# Autodesk Inventor assembly: Inner_Components
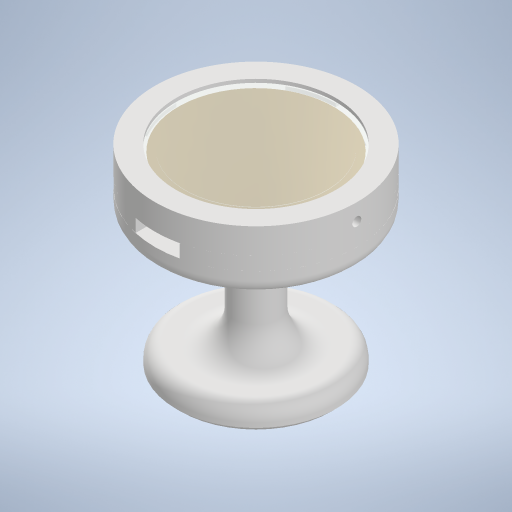
[picture p0: Inventor's stored thumbnail of the model, 512x512]
Saved by Autodesk Inventor 2023 (Build 270158000, 158)
## iProperties
Created: 2023-02-27
Part Number: Inner_Components
Document SubType Name: Assembly
Designer: maste
Author: maste
## Documents named in this file (6)
- C:\Users\maste\Documents\GitHub\Remote-Stethoscope\3D_models\ThonkLabs 1ne\Inner_Components.iam
- C:\Users\maste\Documents\GitHub\Remote-Stethoscope\3D_models\ThonkLabs 1ne\PiezoMount.ipt
- C:\Users\maste\Documents\GitHub\Remote-Stethoscope\3D_models\ThonkLabs 1ne\Piezo.ipt
- C:\Users\maste\Documents\GitHub\Remote-Stethoscope\3D_models\ThonkLabs 1ne\Diaphragm.ipt
- C:\Users\maste\Documents\GitHub\Remote-Stethoscope\3D_models\ThonkLabs 1ne\Diaphragm_lock.ipt
- C:\Users\maste\Documents\GitHub\Remote-Stethoscope\3D_models\ThonkLabs 1ne\holding_socket.ipt
## Components (5 placed, 5 different names)
1. PiezoMount:1 — Mate:1, Mate:2, Mate:3, Mate:4, Mate:6, Mate:7, Mate:8, Mate:9
2. Piezo:1 — Mate:1, Mate:2
3. Diaphragm:1 — Mate:3, Mate:4, Mate:5
4. Diaphragm_lock:1 — Mate:5, Mate:6
5. holding_socket:1 — Mate:7, Mate:8, Mate:9
## Relationships (9: Mate 9)
- Mate:1: PiezoMount:1 ↔ Piezo:1
- Mate:2: PiezoMount:1 ↔ Piezo:1
- Mate:3: PiezoMount:1 ↔ Diaphragm:1
- Mate:4: PiezoMount:1 ↔ Diaphragm:1
- Mate:5: Diaphragm:1 ↔ Diaphragm_lock:1
- Mate:6: PiezoMount:1 ↔ Diaphragm_lock:1
- Mate:7: PiezoMount:1 ↔ holding_socket:1
- Mate:8: PiezoMount:1 ↔ holding_socket:1
- Mate:9: PiezoMount:1 ↔ holding_socket:1
